# Autodesk Inventor assembly: build
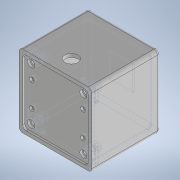
[picture p0: Inventor's stored thumbnail of the model, 180x180]
Saved by Autodesk Inventor 2020 (Build 240168000, 168)
## iProperties
Created: 2022-08-25
Part Number: build
Document SubType Name: Assembly
Designer: zigma
Author: zigma
## Documents named in this file (4)
- C:\Users\zigma\Documents\Work\gitlab_lamp\build.iam
- C:\Users\zigma\Documents\Work\gitlab_lamp\bottom.ipt
- C:\Users\zigma\Documents\Work\gitlab_lamp\box.ipt
- C:\Users\zigma\Documents\Work\gitlab_lamp\holder.ipt
## Components (6 placed, 3 different names)
1. bottom:1 — Совмещение:7, Вставка:1, Вставка:2
2. box:1 — Совмещение:1, Совмещение:2, Совмещение:3, Совмещение:4, Совмещение:5, Совмещение:6
3. holder:1 — Заподлицо:2, Заподлицо:6, Совмещение:5
4. holder:2 — Заподлицо:1, Заподлицо:3, Заподлицо:5, Совмещение:6
5. holder:3 — Заподлицо:1, Заподлицо:4, Заподлицо:5, Совмещение:4, Вставка:2
6. holder:4 — Заподлицо:2, Заподлицо:3, Совмещение:1, Заподлицо:4, Заподлицо:6, Совмещение:2, Совмещение:3, Совмещение:7, Вставка:1
## Relationships (15: Mate 7, Flush 6, Insert 2)
- Заподлицо:1 [Flush]: holder:2 ↔ holder:3
- Заподлицо:2 [Flush]: holder:1 ↔ holder:4
- Заподлицо:3 [Flush]: holder:2 ↔ holder:4
- Совмещение:1 [Mate]: box:1 ↔ holder:4
- Заподлицо:4 [Flush]: holder:3 ↔ holder:4
- Заподлицо:5 [Flush]: holder:2 ↔ holder:3
- Заподлицо:6 [Flush]: holder:1 ↔ holder:4
- Совмещение:2 [Mate]: box:1 ↔ holder:4
- Совмещение:3 [Mate]: box:1 ↔ holder:4
- Совмещение:4 [Mate]: box:1 ↔ holder:3
- Совмещение:5 [Mate]: box:1 ↔ holder:1
- Совмещение:6 [Mate]: box:1 ↔ holder:2
- Совмещение:7 [Mate]: bottom:1 ↔ holder:4
- Вставка:1 [Insert]: bottom:1 ↔ holder:4
- Вставка:2 [Insert]: bottom:1 ↔ holder:3
